# Autodesk Inventor assembly: Stewart-Head
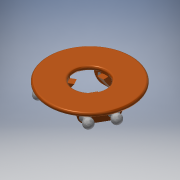
[picture p0: Inventor's stored thumbnail of the model, 180x180]
Saved by Autodesk Inventor 2018.2 (Build 222227000, 227)
## iProperties
Created: 2018-02-23
Part Number: Stewart-Head
Material: Generisch
Document SubType Name: Assembly
Designer: JochenAlt
Author: JochenAlt
## Documents named in this file (3)
- D:\Projects\Donna\CAD\Stewart-Head.iam
- D:\Projects\Donna\CAD\Stewart-Plate-Head.ipt
- D:\Projects\Donna\CAD\Ball-Joint-male.ipt
## Components (7 placed, 2 different names)
1. Stewart-Plate-Head:1 — Passend:1, Passend:2, Passend:3, Passend:4, Passend:5, Passend:6, Passend:7, Passend:8, Passend:9, Passend:10, Passend:11, Passend:12
2. ball joint:1 — Passend:1, Passend:10
3. ball joint:2 — Passend:5, Passend:11
4. ball joint:3 — Passend:6, Passend:12
5. ball joint:4 — Passend:4, Passend:7
6. ball joint:5 — Passend:3, Passend:8
7. ball joint:6 — Passend:2, Passend:9
## Relationships (12: Mate 12)
- Passend:1 [Mate]: Stewart-Plate-Head:1 ↔ ball joint:1
- Passend:2 [Mate]: Stewart-Plate-Head:1 ↔ ball joint:6
- Passend:3 [Mate]: Stewart-Plate-Head:1 ↔ ball joint:5
- Passend:4 [Mate]: Stewart-Plate-Head:1 ↔ ball joint:4
- Passend:5 [Mate]: Stewart-Plate-Head:1 ↔ ball joint:2
- Passend:6 [Mate]: Stewart-Plate-Head:1 ↔ ball joint:3
- Passend:7 [Mate]: Stewart-Plate-Head:1 ↔ ball joint:4
- Passend:8 [Mate]: Stewart-Plate-Head:1 ↔ ball joint:5
- Passend:9 [Mate]: Stewart-Plate-Head:1 ↔ ball joint:6
- Passend:10 [Mate]: Stewart-Plate-Head:1 ↔ ball joint:1
- Passend:11 [Mate]: Stewart-Plate-Head:1 ↔ ball joint:2
- Passend:12 [Mate]: Stewart-Plate-Head:1 ↔ ball joint:3
